# Autodesk Inventor assembly: Rahmen_Seite
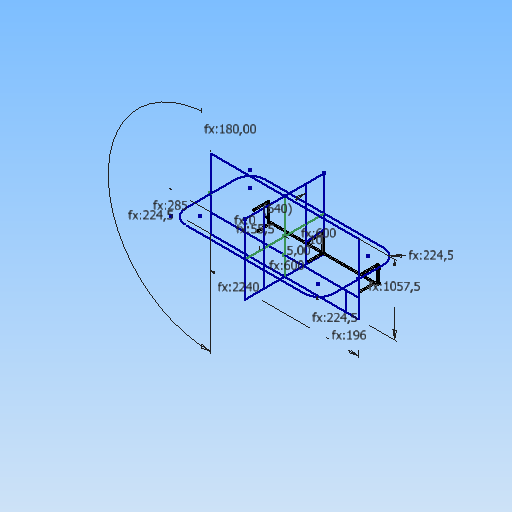
[picture p0: Inventor's stored thumbnail of the model, 512x512]
Saved by Autodesk Inventor 2019.4 (Build 234330000, 330)
## iProperties
Created: 2018-01-19
Part Number: Rahmen_Seite
Material: Generisch
Document SubType Name: Assembly
Designer: hagen
Mass: 2303.54 g
Surface Area: 5729.5 cm^2
Volume: 291.587 cm^3
Density: 7.9 g/cm^3
Stock Number: 2007.006-01.01-200
Description: Rahmen_Seite1
Masse: 43.59 kg
Abmasse: 2240 mm x 720 mm x 1058.5 mm
Author: hagen
## Documents named in this file (9)
- P:\_K\K2017129_e17536_JvK_Fahrradwaschanlage_cycleWASH\Konstruktion_19\DUO Anlage\Gestell\Rahmen_Seite.iam
- P:\_K\K2017129_e17536_JvK_Fahrradwaschanlage_cycleWASH\Konstruktion_19\Parameter Skizze.ipt
- P:\_K\K2017129_e17536_JvK_Fahrradwaschanlage_cycleWASH\Konstruktion_19\DUO Anlage\Gestell\DIN EN 10305-5 - Seitenträger1.ipt
- DIN EN 10305-5 - Träger 2 Breite1.ipt
- P:\_K\K2017129_e17536_JvK_Fahrradwaschanlage_cycleWASH\Konstruktion_19\DUO Anlage\Gestell\DIN EN 10305-5 - Seitenträger2.ipt
- P:\_K\K2017129_e17536_JvK_Fahrradwaschanlage_cycleWASH\Konstruktion_19\DUO Anlage\Gestell\DIN EN 10305-5 - Seitenträger3.ipt
- P:\_K\K2017129_e17536_JvK_Fahrradwaschanlage_cycleWASH\Konstruktion_19\DUO Anlage\Gestell\Lasche1.ipt
- P:\_K\K2017129_e17536_JvK_Fahrradwaschanlage_cycleWASH\Konstruktion_19\DUO Anlage\Gestell\DIN EN 10305-5 - Seitenträger1-gebohrt.ipt
- P:\_K\K2017129_e17536_JvK_Fahrradwaschanlage_cycleWASH\Konstruktion_19\Zukaufteile\KVT\M6_geschlossen\KVT_KVTM6RCROKSG15115\KVT M6 RC ROKSG 1,5 (11_5).ipt
## Components (18 placed, 4 different names)
1. Parameter Skizze.ipt:1 — Fluchtend:49, Fluchtend:50, Fluchtend:51, Passend:1
2. DIN EN 10305-5 - Träger 2 Breite1:1 — Passend:1, Passend:2, Fluchtend:52, Fluchtend:53, Symmetrie:1, Passend:6, Fluchtend:61, Passend:10, Passend:15
3. DIN EN 10305-5 - Träger 2 Breite1:2 — Fluchtend:52, Fluchtend:53, Symmetrie:1, Passend:10
4. DIN EN 10305-5 - Träger 2 Breite1:14 — Fluchtend:55, Passend:16, Fluchtend:89, Passend:20, Fluchtend:90, Einfügen:1
5. DIN EN 10305-5 - Träger 2 Breite1:13 — Fluchtend:55, Fluchtend:87, Fluchtend:88, Einfügen:3
6. DIN EN 10305-5 - Träger 2 Breite1:6 — Passend:5, Passend:6, Fluchtend:61, Passend:7, Fluchtend:63, Fluchtend:64, Fluchtend:67, Fluchtend:68, Passend:8, Passend:19
7. DIN EN 10305-5 - Träger 2 Breite1:7 — Passend:7, Fluchtend:63, Fluchtend:64, Fluchtend:65, Fluchtend:66, Fluchtend:80, Passend:12, Passend:16, Fluchtend:89, Fluchtend:90
8. DIN EN 10305-5 - Träger 2 Breite1:8 — Fluchtend:65, Fluchtend:66, Fluchtend:67, Passend:13, Fluchtend:85, Fluchtend:87, Fluchtend:88
9. DIN EN 10305-5 - Träger 2 Breite1:9 — Fluchtend:68, Passend:8, Fluchtend:69, Fluchtend:71, Fluchtend:81, Fluchtend:84
10. DIN EN 10305-5 - Träger 2 Breite1:12 — Fluchtend:71, Fluchtend:81, Fluchtend:86, Passend:18, Einfügen:2
11. Lasche1:1 — Fluchtend:73, Fluchtend:75, Fluchtend:79, Passend:13
12. Lasche1:2 — Fluchtend:74, Fluchtend:76, Fluchtend:79
13. Lasche1:3 — Fluchtend:73, Fluchtend:75, Fluchtend:77, Fluchtend:78, Fluchtend:80, Passend:12, Passend:20
14. Lasche1:4 — Fluchtend:74, Fluchtend:76, Fluchtend:77, Fluchtend:78, Passend:15
15. DIN EN 10305-5 - Träger 2 Breite1:11 — Fluchtend:84, Fluchtend:85, Fluchtend:86, Passend:18, Passend:19
16. KVT M6 RC ROKSG 1,5 (11_5):1 — Einfügen:1
17. KVT M6 RC ROKSG 1,5 (11_5):2 — Einfügen:2
18. KVT M6 RC ROKSG 1,5 (11_5):3 — Einfügen:3
## Relationships (49: Flush 31, Mate 14, Insert 3, Symmetry 1)
- Fluchtend:49 [Flush]: Parameter Skizze.ipt:1
- Fluchtend:50 [Flush]: Parameter Skizze.ipt:1
- Fluchtend:51 [Flush]: Parameter Skizze.ipt:1
- Passend:1 [Mate]: Parameter Skizze.ipt:1 ↔ DIN EN 10305-5 - Träger 2 Breite1:1
- Passend:2 [Mate] (360 mm): DIN EN 10305-5 - Träger 2 Breite1:1
- Fluchtend:52 [Flush]: DIN EN 10305-5 - Träger 2 Breite1:1 ↔ DIN EN 10305-5 - Träger 2 Breite1:2
- Fluchtend:53 [Flush]: DIN EN 10305-5 - Träger 2 Breite1:1 ↔ DIN EN 10305-5 - Träger 2 Breite1:2
- Fluchtend:55 [Flush]: DIN EN 10305-5 - Träger 2 Breite1:14 ↔ DIN EN 10305-5 - Träger 2 Breite1:13
- Symmetrie:1: DIN EN 10305-5 - Träger 2 Breite1:1 ↔ DIN EN 10305-5 - Träger 2 Breite1:2
- Passend:5 [Mate]: DIN EN 10305-5 - Träger 2 Breite1:6
- Passend:6 [Mate]: DIN EN 10305-5 - Träger 2 Breite1:1 ↔ DIN EN 10305-5 - Träger 2 Breite1:6
- Fluchtend:61 [Flush]: DIN EN 10305-5 - Träger 2 Breite1:1 ↔ DIN EN 10305-5 - Träger 2 Breite1:6
- Passend:7 [Mate]: DIN EN 10305-5 - Träger 2 Breite1:6 ↔ DIN EN 10305-5 - Träger 2 Breite1:7
- Fluchtend:63 [Flush]: DIN EN 10305-5 - Träger 2 Breite1:6 ↔ DIN EN 10305-5 - Träger 2 Breite1:7
- Fluchtend:64 [Flush]: DIN EN 10305-5 - Träger 2 Breite1:6 ↔ DIN EN 10305-5 - Träger 2 Breite1:7
- Fluchtend:65 [Flush]: DIN EN 10305-5 - Träger 2 Breite1:7 ↔ DIN EN 10305-5 - Träger 2 Breite1:8
- Fluchtend:66 [Flush]: DIN EN 10305-5 - Träger 2 Breite1:7 ↔ DIN EN 10305-5 - Träger 2 Breite1:8
- Fluchtend:67 [Flush]: DIN EN 10305-5 - Träger 2 Breite1:6 ↔ DIN EN 10305-5 - Träger 2 Breite1:8
- Fluchtend:68 [Flush]: DIN EN 10305-5 - Träger 2 Breite1:6 ↔ DIN EN 10305-5 - Träger 2 Breite1:9
- Passend:8 [Mate]: DIN EN 10305-5 - Träger 2 Breite1:6 ↔ DIN EN 10305-5 - Träger 2 Breite1:9
- Fluchtend:69 [Flush]: DIN EN 10305-5 - Träger 2 Breite1:9
- Passend:10 [Mate] (-1591 mm): DIN EN 10305-5 - Träger 2 Breite1:1 ↔ DIN EN 10305-5 - Träger 2 Breite1:2
- Fluchtend:71 [Flush]: DIN EN 10305-5 - Träger 2 Breite1:9 ↔ DIN EN 10305-5 - Träger 2 Breite1:12
- Fluchtend:73 [Flush]: Lasche1:1 ↔ Lasche1:3
- Fluchtend:74 [Flush]: Lasche1:2 ↔ Lasche1:4
- Fluchtend:75 [Flush]: Lasche1:1 ↔ Lasche1:3
- Fluchtend:76 [Flush]: Lasche1:2 ↔ Lasche1:4
- Fluchtend:77 [Flush]: Lasche1:3 ↔ Lasche1:4
- Fluchtend:78 [Flush]: Lasche1:3 ↔ Lasche1:4
- Fluchtend:79 [Flush]: Lasche1:1 ↔ Lasche1:2
- Fluchtend:80 [Flush] (6 mm): DIN EN 10305-5 - Träger 2 Breite1:7 ↔ Lasche1:3
- Passend:12 [Mate]: DIN EN 10305-5 - Träger 2 Breite1:7 ↔ Lasche1:3
- Passend:13 [Mate]: DIN EN 10305-5 - Träger 2 Breite1:8 ↔ Lasche1:1
- Passend:15 [Mate] (10 mm): DIN EN 10305-5 - Träger 2 Breite1:1 ↔ Lasche1:4
- Fluchtend:81 [Flush]: DIN EN 10305-5 - Träger 2 Breite1:9 ↔ DIN EN 10305-5 - Träger 2 Breite1:12
- Fluchtend:84 [Flush]: DIN EN 10305-5 - Träger 2 Breite1:9 ↔ DIN EN 10305-5 - Träger 2 Breite1:11
- Fluchtend:85 [Flush]: DIN EN 10305-5 - Träger 2 Breite1:8 ↔ DIN EN 10305-5 - Träger 2 Breite1:11
- Fluchtend:86 [Flush]: DIN EN 10305-5 - Träger 2 Breite1:12 ↔ DIN EN 10305-5 - Träger 2 Breite1:11
- Passend:16 [Mate]: DIN EN 10305-5 - Träger 2 Breite1:14 ↔ DIN EN 10305-5 - Träger 2 Breite1:7
- Fluchtend:87 [Flush]: DIN EN 10305-5 - Träger 2 Breite1:13 ↔ DIN EN 10305-5 - Träger 2 Breite1:8
- Fluchtend:88 [Flush]: DIN EN 10305-5 - Träger 2 Breite1:13 ↔ DIN EN 10305-5 - Träger 2 Breite1:8
- Passend:18 [Mate]: DIN EN 10305-5 - Träger 2 Breite1:12 ↔ DIN EN 10305-5 - Träger 2 Breite1:11
- Passend:19 [Mate]: DIN EN 10305-5 - Träger 2 Breite1:6 ↔ DIN EN 10305-5 - Träger 2 Breite1:11
- Fluchtend:89 [Flush]: DIN EN 10305-5 - Träger 2 Breite1:14 ↔ DIN EN 10305-5 - Träger 2 Breite1:7
- Passend:20 [Mate] (10 mm): DIN EN 10305-5 - Träger 2 Breite1:14 ↔ Lasche1:3
- Fluchtend:90 [Flush]: DIN EN 10305-5 - Träger 2 Breite1:14 ↔ DIN EN 10305-5 - Träger 2 Breite1:7
- Einfügen:1 [Insert]: DIN EN 10305-5 - Träger 2 Breite1:14 ↔ KVT M6 RC ROKSG 1,5 (11_5):1
- Einfügen:2 [Insert]: DIN EN 10305-5 - Träger 2 Breite1:12 ↔ KVT M6 RC ROKSG 1,5 (11_5):2
- Einfügen:3 [Insert]: DIN EN 10305-5 - Träger 2 Breite1:13 ↔ KVT M6 RC ROKSG 1,5 (11_5):3
## Named parameters: H1 = 1057.5 mm, L = 2240 mm, HB = 600 mm, hw = 285 mm, d = 640 mm, rs = 224.5 mm, rw = 0 mm, bs = 0.8 mm, NMT = 40 mm, wst = 1.5 mm, rat = 2.25 mm, nmt2 = 15 mm, wst2 = 1 mm, rat2 = 1.5 mm, le = 196 mm, w = 0 deg
